# Autodesk Inventor assembly: Drive
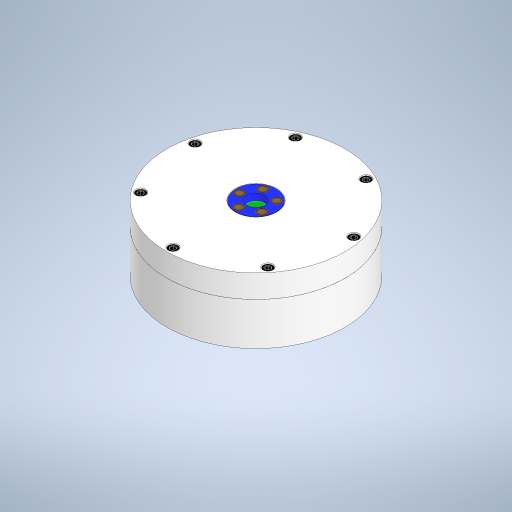
[picture p0: Inventor's stored thumbnail of the model, 512x512]
Saved by Autodesk Inventor 2023 (Build 270158000, 158)
## iProperties
Created: 2023-01-17
Part Number: Drive
Document SubType Name: Assembly
Designer: caden
Author: caden
## Documents named in this file (26)
- C:\Users\caden\OneDrive\Documents\Robotics Club\Cycloidal Drive\Drive.iam
- C:\Users\caden\OneDrive\Documents\Robotics Club\Cycloidal Drive\Epitrochoid.ipt
- C:\Users\caden\OneDrive\Documents\Robotics Club\Cycloidal Drive\Case.ipt
- C:\Users\caden\OneDrive\Documents\Robotics Club\Cycloidal Drive\177x35x10 bearing.ipt
- C:\Users\caden\OneDrive\Documents\Robotics Club\Cycloidal Drive\Input pin holder.ipt
- C:\Users\caden\OneDrive\Documents\Robotics Club\Cycloidal Drive\15x24x5.ipt
- C:\Users\caden\OneDrive\Documents\Robotics Club\Cycloidal Drive\Shaft-1.ipt
- C:\Users\caden\OneDrive\Documents\Robotics Club\Cycloidal Drive\Shaft-2.ipt
- C:\Users\caden\OneDrive\Documents\Robotics Club\Cycloidal Drive\Shaft-3.ipt
- C:\Users\caden\OneDrive\Documents\Robotics Club\Cycloidal Drive\Shaft-4.ipt
- C:\Users\caden\OneDrive\Documents\Robotics Club\Cycloidal Drive\output pin holder.ipt
- C:\Users\caden\OneDrive\Documents\Robotics Club\Cycloidal Drive\91290A252_Steel Socket Head Screw.ipt
- C:\Users\caden\OneDrive\Documents\Robotics Club\Cycloidal Drive\94180A361_ Heat-Set.ipt
- C:\Users\caden\OneDrive\Documents\Robotics Club\Cycloidal Drive\6x13x5 Bearings.ipt
- C:\Users\caden\OneDrive\Documents\Robotics Club\Cycloidal Drive\1mm-spacer.ipt
- C:\Users\caden\OneDrive\Documents\Robotics Club\Cycloidal Drive\9mm-spacer.ipt
- C:\Users\caden\OneDrive\Documents\Robotics Club\Cycloidal Drive\6mm-spacer.ipt
- C:\Users\caden\OneDrive\Documents\Robotics Club\Cycloidal Drive\Pin.ipt
- C:\Users\caden\OneDrive\Documents\Robotics Club\Cycloidal Drive\Lid Case.ipt
- C:\Users\caden\OneDrive\Documents\Robotics Club\Cycloidal Drive\91290A242_m5x20_Alloy Steel Socket Head Screw.ipt
- C:\Users\caden\OneDrive\Documents\Robotics Club\Cycloidal Drive\Motor Adapter.ipt
- C:\Users\caden\OneDrive\Documents\Robotics Club\Cycloidal Drive\94180A331_m3_ Heat-Set Inserts.ipt
- C:\Users\caden\OneDrive\Documents\Robotics Club\Cycloidal Drive\Motor-mount.ipt
- C:\Users\caden\OneDrive\Documents\Robotics Club\Cycloidal Drive\91290A110_m3x5_Alloy Steel Socket Head Screw.ipt
- C:\Users\caden\OneDrive\Documents\Robotics Club\Cycloidal Drive\Connecting pins.ipt
- C:\Users\caden\OneDrive\Documents\Robotics Club\Cycloidal Drive\3D-roller.ipt
## Components (205 placed, 25 different names)
1. Case bottom:1 — Rotational:1, Mate:22, Mate:23, Mate:24, Flush:3, Mate:50, Mate:53, Mate:60, Mate:61, Mate:62, Mate:63
2. 177x35x10 bearing:1 — Rotational:1, Mate:1, Mate:2
3. Input pin holder:1 — Mate:1, Mate:2, Rotational:2, Mate:14, Mate:15, Mate:16
4. Shaft-1:1 — Mate:3, Mate:4, Mate:5, Mate:6, Mate:7, Mate:29, Mate:38, Mate:39, Mate:40
5. Shaft-2:1 — Mate:5, Mate:6, Mate:7, Rotational:3, Mate:26, Mate:27, Mate:28
6. Shaft-3:1 — Mate:26, Mate:27, Mate:28, Mate:29, Rotational:10, Mate:34, Mate:35, Mate:36
7. Shaft-4:1 — Mate:34, Mate:35, Mate:36, Rotational:14, Mate:58, Flush:6, Mate:59, Flush:7
8. 15x24x5:4 — Rotational:2, Mate:3, Mate:4
9. Epitrochoid:1 — Rotational:9, Transitional:1
10. 15x24x5:1 — Rotational:14, Rotational:15
11. 15x24x5:2 — Rotational:10, Rotational:12
12. 15x24x5:3 — Rotational:3, Rotational:9
13. Epitrochoid:2 — Rotational:12, Transitional:2, Transitional:3
14. output pin holder:1 — Rotational:15, Mate:37, Flush:4, Mate:56, Flush:5, Mate:57, Rotational:16
15. Lid Case:1 — Mate:53, Mate:54, Mate:55, Mate:63
16. Motor Adapter:1 — Mate:38, Mate:39, Mate:40, Flush:1, Mate:41, Flush:2, Mate:42, Mate:43
17. 94180A331_m3_ Heat-Set Inserts:1 — Flush:2, Mate:42, Mate:44
18. 94180A331_m3_ Heat-Set Inserts:2 — Flush:1, Mate:41, Mate:45
19. Motor-mount:1 — Mate:43, Mate:44, Mate:45, Mate:46, Mate:47, Mate:48, Mate:49
20. 91290A110_m3x5_Alloy Steel Socket Head Screw:1 — Mate:48, Mate:49
21. 91290A110_m3x5_Alloy Steel Socket Head Screw:2 — Mate:46, Mate:47
22. Connecting pins:1 — Mate:58, Flush:6
23. Connecting pins:3 — Mate:59, Flush:7
24. 177x35x10 bearing:2 — Rotational:16
25. 94180A361_ Heat-Set:7 — Flush:5, Mate:57
26. 91290A252_Steel Socket Head Screw:1 — Mate:14, Mate:15, Mate:17, Mate:31, Mate:37
27. 6x13x5 Bearings:1 — Rotational:11, Transitional:2, Transitional:3
28. 6mm-spacer:22 — Mate:30, Mate:31, Rotational:11
29. 6x13x5 Bearings:7 — Rotational:6, Transitional:1, Mate:30
30. 1mm-spacer:1 — Mate:16, Mate:17, Rotational:6
31. 94180A361_ Heat-Set:15
32. 91290A252_Steel Socket Head Screw:2
33. 6x13x5 Bearings:8
34. 6mm-spacer:23
35. 6x13x5 Bearings:9
36. 1mm-spacer:2
37. 94180A361_ Heat-Set:16
38. 91290A252_Steel Socket Head Screw:3
39. 6x13x5 Bearings:10
40. 6mm-spacer:24
41. 6x13x5 Bearings:11
42. 1mm-spacer:3
43. 94180A361_ Heat-Set:17
44. 91290A252_Steel Socket Head Screw:4
45. 6x13x5 Bearings:12
46. 6mm-spacer:25
47. 6x13x5 Bearings:13
48. 1mm-spacer:4
49. 94180A361_ Heat-Set:18
50. 91290A252_Steel Socket Head Screw:5
51. 6x13x5 Bearings:14
52. 6mm-spacer:26
53. 6x13x5 Bearings:15
54. 1mm-spacer:5
55. 94180A361_ Heat-Set:19
56. 91290A252_Steel Socket Head Screw:6
57. 6x13x5 Bearings:16
58. 6mm-spacer:27
59. 6x13x5 Bearings:17
60. 1mm-spacer:6
61. 94180A361_ Heat-Set:14 — Flush:4, Mate:56
62. 94180A361_ Heat-Set:20
63. 94180A361_ Heat-Set:21
64. 94180A361_ Heat-Set:22
65. 94180A361_ Heat-Set:23
66. 91290A242_m5x20_Alloy Steel Socket Head Screw:1 — Mate:54, Mate:55
67. 94180A361_ Heat-Set:1 — Flush:3, Mate:50
68. 91290A242_m5x20_Alloy Steel Socket Head Screw:2
69. 94180A361_ Heat-Set:24
70. 91290A242_m5x20_Alloy Steel Socket Head Screw:3
71. 94180A361_ Heat-Set:25
72. 91290A242_m5x20_Alloy Steel Socket Head Screw:4 — Mate:62
73. 94180A361_ Heat-Set:26
74. 91290A242_m5x20_Alloy Steel Socket Head Screw:5
75. 94180A361_ Heat-Set:27
76. 91290A242_m5x20_Alloy Steel Socket Head Screw:6
77. 94180A361_ Heat-Set:28
78. 91290A242_m5x20_Alloy Steel Socket Head Screw:7
79. 94180A361_ Heat-Set:29
80. Pin:1 — Mate:22, Mate:23, Mate:25, Mate:33
81. 9mm-spacer:1 — Mate:24, Mate:25, Rotational:17
82. 6x13x5 Bearings:19 — Rotational:17
83. 6mm-spacer:1 — Mate:33, Rotational:18
84. 6x13x5 Bearings:20 — Rotational:18
85. Pin:2
86. 9mm-spacer:2
87. 6x13x5 Bearings:21
88. 6mm-spacer:28
89. 6x13x5 Bearings:22
90. Pin:3
91. 9mm-spacer:3
92. 6x13x5 Bearings:23
93. 6mm-spacer:29
94. 6x13x5 Bearings:24
95. Pin:4
96. 9mm-spacer:4
97. 6x13x5 Bearings:25
98. 6mm-spacer:30
99. 6x13x5 Bearings:26
100. Pin:5
101. 9mm-spacer:5
102. 6x13x5 Bearings:27
103. 6mm-spacer:31
104. 6x13x5 Bearings:28
105. Pin:6
106. 9mm-spacer:6
107. 6x13x5 Bearings:29
108. 6mm-spacer:32
109. 6x13x5 Bearings:30
110. Pin:7
111. 9mm-spacer:7
112. 6x13x5 Bearings:31
113. 6mm-spacer:33
114. 6x13x5 Bearings:32
115. Pin:8
116. 9mm-spacer:8
117. 6x13x5 Bearings:33
118. 6mm-spacer:34
119. 6x13x5 Bearings:34
120. Pin:9
121. 9mm-spacer:9
122. 6x13x5 Bearings:35
123. 6mm-spacer:35
124. 6x13x5 Bearings:36
125. Pin:10
126. 9mm-spacer:10
127. 6x13x5 Bearings:37
128. 6mm-spacer:36
129. 6x13x5 Bearings:38
130. Pin:11
131. 9mm-spacer:11
132. 6x13x5 Bearings:39
133. 6mm-spacer:37
134. 6x13x5 Bearings:40
135. Pin:12
136. 9mm-spacer:12
137. 6x13x5 Bearings:41
138. 6mm-spacer:38
139. 6x13x5 Bearings:42
140. Pin:13
141. 9mm-spacer:13
142. 6x13x5 Bearings:43
143. 6mm-spacer:39
144. 6x13x5 Bearings:44
145. Pin:14
146. 9mm-spacer:14
147. 6x13x5 Bearings:45
148. 6mm-spacer:40
149. 6x13x5 Bearings:46
150. Pin:15
151. 9mm-spacer:15
152. 6x13x5 Bearings:47
153. 6mm-spacer:41
154. 6x13x5 Bearings:48
155. Pin:16
156. 9mm-spacer:16
157. 6x13x5 Bearings:49
158. 6mm-spacer:42
159. 6x13x5 Bearings:50
160. Pin:17
161. 9mm-spacer:17
162. 6x13x5 Bearings:51
163. 6mm-spacer:43
164. 6x13x5 Bearings:52
165. Pin:18
166. 9mm-spacer:18
167. 6x13x5 Bearings:53
168. 6mm-spacer:44
169. 6x13x5 Bearings:54
170. Pin:19
171. 9mm-spacer:19
172. 6x13x5 Bearings:55
173. 6mm-spacer:45
174. 6x13x5 Bearings:56
175. Pin:20
176. 9mm-spacer:20
177. 6x13x5 Bearings:57
178. 6mm-spacer:46
179. 6x13x5 Bearings:58
180. Pin:21
181. 9mm-spacer:21
182. 6x13x5 Bearings:59
183. 6mm-spacer:47
184. 6x13x5 Bearings:60
185. 3D-roller:1 — Mate:60, Mate:61
186. 3D-roller:2
187. 3D-roller:3
188. 3D-roller:4
189. 3D-roller:5
190. 3D-roller:6
191. 3D-roller:7
192. 3D-roller:8
193. 3D-roller:9
194. 3D-roller:10
195. 3D-roller:11
196. 3D-roller:12
197. 3D-roller:13
198. 3D-roller:14
199. 3D-roller:15
200. 3D-roller:16
201. 3D-roller:17
202. 3D-roller:18
203. 3D-roller:19
204. 3D-roller:20
205. 3D-roller:21
## Component patterns: (6 elements, first: 94180A361_ Heat-Set:7 + 91290A252_Steel Socket Head Screw:1 + 6x13x5 Bearings:1 + 6mm-spacer:22 + 6x13x5 Bearings:7 + 1mm-spacer:1), (5 elements, first: 94180A361_ Heat-Set:14), (7 elements, first: 91290A242_m5x20_Alloy Steel Socket Head Screw:1 + 94180A361_ Heat-Set:1), (21 elements, first: Pin:1 + 9mm-spacer:1 + 6x13x5 Bearings:19 + 6mm-spacer:1 + 6x13x5 Bearings:20), (21 elements, first: 3D-roller:1)
## Relationships (73: Mate 50, RevoluteJoint 13, Flush 7, Transitional 3)
- Rotational:1 [RevoluteJoint]: Case bottom:1 ↔ 177x35x10 bearing:1
- Mate:1: 177x35x10 bearing:1 ↔ Input pin holder:1
- Mate:2: 177x35x10 bearing:1 ↔ Input pin holder:1
- Rotational:2 [RevoluteJoint]: Input pin holder:1 ↔ 15x24x5:4
- Mate:3: Shaft-1:1 ↔ 15x24x5:4
- Mate:4: Shaft-1:1 ↔ 15x24x5:4
- Mate:5: Shaft-1:1 ↔ Shaft-2:1
- Mate:6: Shaft-1:1 ↔ Shaft-2:1
- Mate:7: Shaft-1:1 ↔ Shaft-2:1
- Rotational:3 [RevoluteJoint]: Shaft-2:1 ↔ 15x24x5:3
- Mate:14: Input pin holder:1 ↔ 91290A252_Steel Socket Head Screw:1
- Mate:15: Input pin holder:1 ↔ 91290A252_Steel Socket Head Screw:1
- Mate:16: Input pin holder:1 ↔ 1mm-spacer:1
- Mate:17: 91290A252_Steel Socket Head Screw:1 ↔ 1mm-spacer:1
- Rotational:6 [RevoluteJoint]: 6x13x5 Bearings:7 ↔ 1mm-spacer:1
- Mate:22: Case bottom:1 ↔ Pin:1
- Mate:23: Case bottom:1 ↔ Pin:1
- Mate:24: Case bottom:1 ↔ 9mm-spacer:1
- Mate:25: Pin:1 ↔ 9mm-spacer:1
- Rotational:9 [RevoluteJoint]: Epitrochoid:1 ↔ 15x24x5:3
- Transitional:1: Epitrochoid:1 ↔ 6x13x5 Bearings:7
- Mate:26: Shaft-2:1 ↔ Shaft-3:1
- Mate:27: Shaft-2:1 ↔ Shaft-3:1
- Mate:28: Shaft-2:1 ↔ Shaft-3:1
- Mate:29: Shaft-1:1 ↔ Shaft-3:1
- Rotational:10 [RevoluteJoint]: Shaft-3:1 ↔ 15x24x5:2
- Mate:30: 6mm-spacer:22 ↔ 6x13x5 Bearings:7
- Mate:31: 91290A252_Steel Socket Head Screw:1 ↔ 6mm-spacer:22
- Rotational:11 [RevoluteJoint]: 6x13x5 Bearings:1 ↔ 6mm-spacer:22
- Rotational:12 [RevoluteJoint]: 15x24x5:2 ↔ Epitrochoid:2
- Transitional:2: Epitrochoid:2 ↔ 6x13x5 Bearings:1
- Mate:33: Pin:1 ↔ 6mm-spacer:1
- Mate:34: Shaft-3:1 ↔ Shaft-4:1
- Mate:35: Shaft-3:1 ↔ Shaft-4:1
- Mate:36: Shaft-3:1 ↔ Shaft-4:1
- Rotational:14 [RevoluteJoint]: Shaft-4:1 ↔ 15x24x5:1
- Rotational:15 [RevoluteJoint]: 15x24x5:1 ↔ output pin holder:1
- Mate:37: output pin holder:1 ↔ 91290A252_Steel Socket Head Screw:1
- Mate:38: Shaft-1:1 ↔ Motor Adapter:1
- Mate:39: Shaft-1:1 ↔ Motor Adapter:1
- Mate:40: Shaft-1:1 ↔ Motor Adapter:1
- Flush:1: Motor Adapter:1 ↔ 94180A331_m3_ Heat-Set Inserts:2
- Mate:41: Motor Adapter:1 ↔ 94180A331_m3_ Heat-Set Inserts:2
- Flush:2: Motor Adapter:1 ↔ 94180A331_m3_ Heat-Set Inserts:1
- Mate:42: Motor Adapter:1 ↔ 94180A331_m3_ Heat-Set Inserts:1
- Mate:43: Motor Adapter:1 ↔ Motor-mount:1
- Mate:44: 94180A331_m3_ Heat-Set Inserts:1 ↔ Motor-mount:1
- Mate:45: 94180A331_m3_ Heat-Set Inserts:2 ↔ Motor-mount:1
- Mate:46: Motor-mount:1 ↔ 91290A110_m3x5_Alloy Steel Socket Head Screw:2
- Mate:47: Motor-mount:1 ↔ 91290A110_m3x5_Alloy Steel Socket Head Screw:2
- Mate:48: Motor-mount:1 ↔ 91290A110_m3x5_Alloy Steel Socket Head Screw:1
- Mate:49: Motor-mount:1 ↔ 91290A110_m3x5_Alloy Steel Socket Head Screw:1
- Flush:3: Case bottom:1 ↔ 94180A361_ Heat-Set:1
- Mate:50: Case bottom:1 ↔ 94180A361_ Heat-Set:1
- Mate:53: Case bottom:1 ↔ Lid Case:1
- Mate:54: Lid Case:1 ↔ 91290A242_m5x20_Alloy Steel Socket Head Screw:1
- Mate:55: Lid Case:1 ↔ 91290A242_m5x20_Alloy Steel Socket Head Screw:1
- Flush:4: output pin holder:1 ↔ 94180A361_ Heat-Set:14
- Mate:56: output pin holder:1 ↔ 94180A361_ Heat-Set:14
- Flush:5: output pin holder:1 ↔ 94180A361_ Heat-Set:7
- Mate:57: output pin holder:1 ↔ 94180A361_ Heat-Set:7
- Mate:58: Shaft-4:1 ↔ Connecting pins:1
- Flush:6: Shaft-4:1 ↔ Connecting pins:1
- Mate:59: Shaft-4:1 ↔ Connecting pins:3
- Flush:7: Shaft-4:1 ↔ Connecting pins:3
- Rotational:16 [RevoluteJoint]: output pin holder:1 ↔ 177x35x10 bearing:2
- Rotational:17 [RevoluteJoint]: 9mm-spacer:1 ↔ 6x13x5 Bearings:19
- Rotational:18 [RevoluteJoint]: 6mm-spacer:1 ↔ 6x13x5 Bearings:20
- Mate:60: Case bottom:1 ↔ 3D-roller:1
- Mate:61: Case bottom:1 ↔ 3D-roller:1
- Mate:62: Case bottom:1 ↔ 91290A242_m5x20_Alloy Steel Socket Head Screw:4
- Mate:63: Case bottom:1 ↔ Lid Case:1
- Transitional:3: Epitrochoid:2 ↔ 6x13x5 Bearings:1
